(part 1 of 2)
# Autodesk Inventor assembly: Functioning Test Chasis
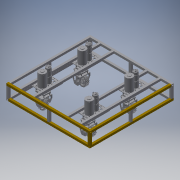
[picture p0: Inventor's stored thumbnail of the model, 180x180]
Saved by Autodesk Inventor 2019 (Build 230136000, 136)
## iProperties
has-driver: True
driver-type: 1
motor-type: 0
driver-port1: 0
driver-port2: -1
driver-isCan: False
driver-lowerLimit: 0.0
driver-upperLimit: 0.0
driver-inputGear: 0.0
driver-outputGear: 0.0
driver-hasBrake: False
has-wheel: True
wheel-type: 3
wheel-isDriveWheel: True
wheel-frictionLevel: 1
has-pneumatic: False
has-elevator: False
num-sensors: 0
has-driver: False
driver-port1: 1
robot-name: Chasis
robot-weight-kg: 222.26052856445312
robot-prefer-metric: False
robot-driveTrainType: 1
Created: 2019-01-14
Part Number: Functioning Test Chasis
Document SubType Name: Assembly
Designer: josh
Author: josh
## Documents named in this file (37)
- D:\Synthesis Robots\Epsilon\Functioning Test Chasis.iam
- D:\Synthesis Robots\Epsilon\Chasis.iam
- D:\Synthesis Robots\Epsilon\functioning swerve drive.iam
- D:\Synthesis Robots\Epsilon\4 in HiGrip Wheel.iam
- D:\Synthesis Robots\Epsilon\FR6ZZ-L Hex Bearing.ipt
- D:\Synthesis Robots\Epsilon\375 Hex Output Shaft Rev 2.ipt
- D:\Synthesis Robots\Epsilon\375 Hex Hub.ipt
- D:\Synthesis Robots\Epsilon\10-24 Hex Washer Rolling x 3-4_93882A213.ipt
- D:\Synthesis Robots\Epsilon\125x443 spacer SPS-0750-0443-0125.ipt
- D:\Synthesis Robots\Epsilon\375 E-klip - Mcm 97431A320_97431A320.ipt
- D:\Synthesis Robots\Epsilon\20t 1-25mod bevel gear.ipt
- D:\Synthesis Robots\Epsilon\40t 1-25mod bevel gear.ipt
- D:\Synthesis Robots\Epsilon\AMS C Housing Rev 2.ipt
- D:\Synthesis Robots\Epsilon\10-32 Nylock Nut 1_90631A411.ipt
- D:\Synthesis Robots\Epsilon\10-32x1250_shcs.ipt
- D:\Synthesis Robots\Epsilon\620x215 alum spacer 83062 K-S.ipt
- D:\Synthesis Robots\Epsilon\Bevel Input Shaft.ipt
- D:\Synthesis Robots\Epsilon\FR8ZZ Bearing_smart.ipt
- D:\Synthesis Robots\Epsilon\FR6ZZ Bearing_smart.ipt
- D:\Synthesis Robots\Epsilon\12T CIM Shaft.ipt
- D:\Synthesis Robots\Epsilon\Gear Plate.ipt
- D:\Synthesis Robots\Epsilon\40T 20dp 375h_Inch - Spur gear 20DP 40T 14.5PA .372FW ---S40N3.0H2.0L0.25N.ipt
- D:\Synthesis Robots\Epsilon\500 Washer am-1001.ipt
- D:\Synthesis Robots\Epsilon\10-32x0625_shcs_HX-SHCS 0.19-32x1.375x1-C.ipt
- D:\Synthesis Robots\Epsilon\1100x215 alum spacer 83062 K-S.ipt
- D:\Synthesis Robots\Epsilon\10-32 Nylock Nut.ipt
- D:\Synthesis Robots\Epsilon\10-32x1750_shcs_HX-SHCS 0.19-32x1.375x1-C.ipt
- D:\Synthesis Robots\Epsilon\Bearing Plate.ipt
- D:\Synthesis Robots\Epsilon\40T Sleeve Gear REV2.ipt
- D:\Synthesis Robots\Epsilon\VEX 217-2736 0500 Collar Clamp.ipt
- D:\Synthesis Robots\Epsilon\CIM Motor SW.ipt
- D:\Synthesis Robots\Epsilon\Motor Mount Plate Rev 2.ipt
- D:\Synthesis Robots\Epsilon\48T 10mm bore gear.ipt
- D:\Synthesis Robots\Epsilon\PG-71.ipt
- D:\Synthesis Robots\Epsilon\SHCS M4x10_91290A187.ipt
- D:\Synthesis Robots\Epsilon\438x406 spacer 13RS100043.ipt
- D:\Synthesis Robots\Epsilon\375 External Self Locking Ring_98430A134.ipt
## Components (274 placed, 36 different names)
1. Chasis:1 [sub-assembly] — Mate:253, Flush:23, Mate:254, Mate:505, Flush:46, Mate:506, Mate:507, Flush:47, Mate:508, Mate:634, Flush:59, Mate:635
2. functioning swerve drive:1 [sub-assembly]
3. FR6ZZ-L Hex Bearing:3
4. FR6ZZ-L Hex Bearing:4
5. 375 Hex Output Shaft Rev 2:2
6. 375 Hex Hub:2
7. 10-24 Hex Washer Rolling x 3-4_93882A213:7
8. 10-24 Hex Washer Rolling x 3-4_93882A213:8
9. 10-24 Hex Washer Rolling x 3-4_93882A213:9
10. 10-24 Hex Washer Rolling x 3-4_93882A213:10
11. 10-24 Hex Washer Rolling x 3-4_93882A213:11
12. 10-24 Hex Washer Rolling x 3-4_93882A213:12
13. 125x443 spacer SPS-0750-0443-0125:2
14. 375 E-klip - Mcm 97431A320_97431A320:2
15. 20t 1-25mod bevel gear:2
16. 40t 1-25mod bevel gear:2
17. AMS C Housing Rev 2:2
18. 10-32 Nylock Nut 1_90631A411:5
19. 10-32 Nylock Nut 1_90631A411:6
20. 10-32 Nylock Nut 1_90631A411:7
21. 10-32 Nylock Nut 1_90631A411:8
22. 10-32x1250_shcs:5
23. 10-32x1250_shcs:6
24. 10-32x1250_shcs:7
25. 10-32x1250_shcs:8
26. 620x215 alum spacer 83062 K-S:5
27. 620x215 alum spacer 83062 K-S:6
28. 620x215 alum spacer 83062 K-S:7
29. 620x215 alum spacer 83062 K-S:8
30. Bevel Input Shaft:2
31. FR8ZZ Bearing_smart:2
32. FR6ZZ Bearing_smart:3
33. 12T CIM Shaft:2
34. Gear Plate:2
35. 40T 20dp 375h_Inch - Spur gear 20DP 40T 14.5PA .372FW ---S40N3.0H2.0L0.25N:2
36. 500 Washer am-1001:3
37. 500 Washer am-1001:4
38. FR6ZZ Bearing_smart:4
39. 10-32x0625_shcs_HX-SHCS 0.19-32x1.375x1-C:7
40. 10-32x0625_shcs_HX-SHCS 0.19-32x1.375x1-C:8
41. 10-32x0625_shcs_HX-SHCS 0.19-32x1.375x1-C:9
42. 10-32x0625_shcs_HX-SHCS 0.19-32x1.375x1-C:10
43. 1100x215 alum spacer 83062 K-S:5
44. 10-32 Nylock Nut:5
45. 10-32x1750_shcs_HX-SHCS 0.19-32x1.375x1-C:5
46. 1100x215 alum spacer 83062 K-S:6
47. 1100x215 alum spacer 83062 K-S:7
48. 1100x215 alum spacer 83062 K-S:8
49. 10-32x1750_shcs_HX-SHCS 0.19-32x1.375x1-C:6
50. 10-32x1750_shcs_HX-SHCS 0.19-32x1.375x1-C:7
51. 10-32x1750_shcs_HX-SHCS 0.19-32x1.375x1-C:8
52. 10-32 Nylock Nut:6
53. 10-32 Nylock Nut:7
54. 10-32 Nylock Nut:8
55. Bearing Plate:2
56. 40T Sleeve Gear REV2:2
57. VEX 217-2736 0500 Collar Clamp:2
58. CIM Motor SW:2
59. Motor Mount Plate Rev 2:2 — Mate:253, Flush:23, Mate:254
60. 48T 10mm bore gear:2
61. 10-32x0625_shcs_HX-SHCS 0.19-32x1.375x1-C:11
62. 10-32x0625_shcs_HX-SHCS 0.19-32x1.375x1-C:12
63. PG-71:2
64. SHCS M4x10_91290A187:5
65. SHCS M4x10_91290A187:6
66. SHCS M4x10_91290A187:7
67. SHCS M4x10_91290A187:8
68. 438x406 spacer 13RS100043:2
69. 375 External Self Locking Ring_98430A134:2
70. 4 in HiGrip Wheel:2 [sub-assembly]
71. FR6ZZ-L Hex Bearing:5
72. FR6ZZ-L Hex Bearing:6
73. 375 Hex Output Shaft Rev 2:3
74. 375 Hex Hub:3
75. 10-24 Hex Washer Rolling x 3-4_93882A213:13
76. 10-24 Hex Washer Rolling x 3-4_93882A213:14
77. 10-24 Hex Washer Rolling x 3-4_93882A213:15
78. 10-24 Hex Washer Rolling x 3-4_93882A213:16
79. 10-24 Hex Washer Rolling x 3-4_93882A213:17
80. 10-24 Hex Washer Rolling x 3-4_93882A213:18
81. 125x443 spacer SPS-0750-0443-0125:3
82. 375 E-klip - Mcm 97431A320_97431A320:3
83. 20t 1-25mod bevel gear:3
84. 40t 1-25mod bevel gear:3
85. AMS C Housing Rev 2:3
86. 10-32 Nylock Nut 1_90631A411:9
87. 10-32 Nylock Nut 1_90631A411:10
88. 10-32 Nylock Nut 1_90631A411:11
89. 10-32 Nylock Nut 1_90631A411:12
90. 10-32x1250_shcs:9
91. 10-32x1250_shcs:10
92. 10-32x1250_shcs:11
93. 10-32x1250_shcs:12
94. 620x215 alum spacer 83062 K-S:9
95. 620x215 alum spacer 83062 K-S:10
96. 620x215 alum spacer 83062 K-S:11
97. 620x215 alum spacer 83062 K-S:12
98. Bevel Input Shaft:3
99. FR8ZZ Bearing_smart:3
100. FR6ZZ Bearing_smart:5
101. 12T CIM Shaft:3
102. Gear Plate:3
103. 40T 20dp 375h_Inch - Spur gear 20DP 40T 14.5PA .372FW ---S40N3.0H2.0L0.25N:3
104. 500 Washer am-1001:5
105. 500 Washer am-1001:6
106. FR6ZZ Bearing_smart:6
107. 10-32x0625_shcs_HX-SHCS 0.19-32x1.375x1-C:13
108. 10-32x0625_shcs_HX-SHCS 0.19-32x1.375x1-C:14
109. 10-32x0625_shcs_HX-SHCS 0.19-32x1.375x1-C:15
110. 10-32x0625_shcs_HX-SHCS 0.19-32x1.375x1-C:16
111. 1100x215 alum spacer 83062 K-S:9
112. 10-32 Nylock Nut:9
113. 10-32x1750_shcs_HX-SHCS 0.19-32x1.375x1-C:9
114. 1100x215 alum spacer 83062 K-S:10
115. 1100x215 alum spacer 83062 K-S:11
116. 1100x215 alum spacer 83062 K-S:12
117. 10-32x1750_shcs_HX-SHCS 0.19-32x1.375x1-C:10
118. 10-32x1750_shcs_HX-SHCS 0.19-32x1.375x1-C:11
119. 10-32x1750_shcs_HX-SHCS 0.19-32x1.375x1-C:12
120. 10-32 Nylock Nut:10
121. 10-32 Nylock Nut:11
122. 10-32 Nylock Nut:12
123. Bearing Plate:3
124. 40T Sleeve Gear REV2:3
125. VEX 217-2736 0500 Collar Clamp:3
126. CIM Motor SW:3
127. Motor Mount Plate Rev 2:3 — Mate:505, Flush:46, Mate:506
128. 48T 10mm bore gear:3
129. 10-32x0625_shcs_HX-SHCS 0.19-32x1.375x1-C:17
130. 10-32x0625_shcs_HX-SHCS 0.19-32x1.375x1-C:18
131. PG-71:3
132. SHCS M4x10_91290A187:9
133. SHCS M4x10_91290A187:10
134. SHCS M4x10_91290A187:11
135. SHCS M4x10_91290A187:12
136. 438x406 spacer 13RS100043:3
137. 375 External Self Locking Ring_98430A134:3
138. 4 in HiGrip Wheel:3 [sub-assembly]
139. FR6ZZ-L Hex Bearing:7
140. FR6ZZ-L Hex Bearing:8
141. 375 Hex Output Shaft Rev 2:4
142. 375 Hex Hub:4
143. 10-24 Hex Washer Rolling x 3-4_93882A213:19
144. 10-24 Hex Washer Rolling x 3-4_93882A213:20
145. 10-24 Hex Washer Rolling x 3-4_93882A213:21
146. 10-24 Hex Washer Rolling x 3-4_93882A213:22
147. 10-24 Hex Washer Rolling x 3-4_93882A213:23
148. 10-24 Hex Washer Rolling x 3-4_93882A213:24
149. 125x443 spacer SPS-0750-0443-0125:4
150. 375 E-klip - Mcm 97431A320_97431A320:4
151. 20t 1-25mod bevel gear:4
152. 40t 1-25mod bevel gear:4
153. AMS C Housing Rev 2:4
154. 10-32 Nylock Nut 1_90631A411:13
155. 10-32 Nylock Nut 1_90631A411:14
156. 10-32 Nylock Nut 1_90631A411:15
157. 10-32 Nylock Nut 1_90631A411:16
158. 10-32x1250_shcs:13
159. 10-32x1250_shcs:14
160. 10-32x1250_shcs:15
161. 10-32x1250_shcs:16
162. 620x215 alum spacer 83062 K-S:13
163. 620x215 alum spacer 83062 K-S:14
164. 620x215 alum spacer 83062 K-S:15
165. 620x215 alum spacer 83062 K-S:16
166. Bevel Input Shaft:4
167. FR8ZZ Bearing_smart:4
168. FR6ZZ Bearing_smart:7
169. 12T CIM Shaft:4
170. Gear Plate:4
171. 40T 20dp 375h_Inch - Spur gear 20DP 40T 14.5PA .372FW ---S40N3.0H2.0L0.25N:4
172. 500 Washer am-1001:7
173. 500 Washer am-1001:8
174. FR6ZZ Bearing_smart:8
175. 10-32x0625_shcs_HX-SHCS 0.19-32x1.375x1-C:19
176. 10-32x0625_shcs_HX-SHCS 0.19-32x1.375x1-C:20
177. 10-32x0625_shcs_HX-SHCS 0.19-32x1.375x1-C:21
178. 10-32x0625_shcs_HX-SHCS 0.19-32x1.375x1-C:22
179. 1100x215 alum spacer 83062 K-S:13
180. 10-32 Nylock Nut:13
181. 10-32x1750_shcs_HX-SHCS 0.19-32x1.375x1-C:13
182. 1100x215 alum spacer 83062 K-S:14
183. 1100x215 alum spacer 83062 K-S:15
184. 1100x215 alum spacer 83062 K-S:16
185. 10-32x1750_shcs_HX-SHCS 0.19-32x1.375x1-C:14
186. 10-32x1750_shcs_HX-SHCS 0.19-32x1.375x1-C:15
187. 10-32x1750_shcs_HX-SHCS 0.19-32x1.375x1-C:16
188. 10-32 Nylock Nut:14
189. 10-32 Nylock Nut:15
190. 10-32 Nylock Nut:16
191. Bearing Plate:4
192. 40T Sleeve Gear REV2:4
193. VEX 217-2736 0500 Collar Clamp:4
194. CIM Motor SW:4
195. Motor Mount Plate Rev 2:4 — Mate:507, Flush:47, Mate:508
196. 48T 10mm bore gear:4
197. 10-32x0625_shcs_HX-SHCS 0.19-32x1.375x1-C:23
198. 10-32x0625_shcs_HX-SHCS 0.19-32x1.375x1-C:24
199. PG-71:4
200. SHCS M4x10_91290A187:13
201. SHCS M4x10_91290A187:14
202. SHCS M4x10_91290A187:15
203. SHCS M4x10_91290A187:16
204. 438x406 spacer 13RS100043:4
205. 375 External Self Locking Ring_98430A134:4
206. 4 in HiGrip Wheel:4 [sub-assembly]
207. FR6ZZ-L Hex Bearing:9
208. FR6ZZ-L Hex Bearing:10
209. 375 Hex Output Shaft Rev 2:5
210. 375 Hex Hub:5
211. 10-24 Hex Washer Rolling x 3-4_93882A213:25
212. 10-24 Hex Washer Rolling x 3-4_93882A213:26
213. 10-24 Hex Washer Rolling x 3-4_93882A213:27
214. 10-24 Hex Washer Rolling x 3-4_93882A213:28
215. 10-24 Hex Washer Rolling x 3-4_93882A213:29
216. 10-24 Hex Washer Rolling x 3-4_93882A213:30
217. 125x443 spacer SPS-0750-0443-0125:5
218. 375 E-klip - Mcm 97431A320_97431A320:5
219. 20t 1-25mod bevel gear:5
220. 40t 1-25mod bevel gear:5
221. AMS C Housing Rev 2:5
222. 10-32 Nylock Nut 1_90631A411:17
223. 10-32 Nylock Nut 1_90631A411:18
224. 10-32 Nylock Nut 1_90631A411:19
225. 10-32 Nylock Nut 1_90631A411:20
226. 10-32x1250_shcs:17
227. 10-32x1250_shcs:18
228. 10-32x1250_shcs:19
229. 10-32x1250_shcs:20
230. 620x215 alum spacer 83062 K-S:17
231. 620x215 alum spacer 83062 K-S:18
232. 620x215 alum spacer 83062 K-S:19
233. 620x215 alum spacer 83062 K-S:20
234. Bevel Input Shaft:5
235. FR8ZZ Bearing_smart:5
236. FR6ZZ Bearing_smart:9
237. 12T CIM Shaft:5
238. Gear Plate:5
239. 40T 20dp 375h_Inch - Spur gear 20DP 40T 14.5PA .372FW ---S40N3.0H2.0L0.25N:5
240. 500 Washer am-1001:9
241. 500 Washer am-1001:10
242. FR6ZZ Bearing_smart:10
243. 10-32x0625_shcs_HX-SHCS 0.19-32x1.375x1-C:25
244. 10-32x0625_shcs_HX-SHCS 0.19-32x1.375x1-C:26
245. 10-32x0625_shcs_HX-SHCS 0.19-32x1.375x1-C:27
246. 10-32x0625_shcs_HX-SHCS 0.19-32x1.375x1-C:28
247. 1100x215 alum spacer 83062 K-S:17
248. 10-32 Nylock Nut:17
249. 10-32x1750_shcs_HX-SHCS 0.19-32x1.375x1-C:17
250. 1100x215 alum spacer 83062 K-S:18
251. 1100x215 alum spacer 83062 K-S:19
252. 1100x215 alum spacer 83062 K-S:20
253. 10-32x1750_shcs_HX-SHCS 0.19-32x1.375x1-C:18
254. 10-32x1750_shcs_HX-SHCS 0.19-32x1.375x1-C:19
255. 10-32x1750_shcs_HX-SHCS 0.19-32x1.375x1-C:20
256. 10-32 Nylock Nut:18
257. 10-32 Nylock Nut:19
258. 10-32 Nylock Nut:20
259. Bearing Plate:5
260. 40T Sleeve Gear REV2:5
261. VEX 217-2736 0500 Collar Clamp:5
262. CIM Motor SW:5
263. Motor Mount Plate Rev 2:5 — Mate:634, Flush:59, Mate:635
264. 48T 10mm bore gear:5
265. 10-32x0625_shcs_HX-SHCS 0.19-32x1.375x1-C:29
266. 10-32x0625_shcs_HX-SHCS 0.19-32x1.375x1-C:30
267. PG-71:5
268. SHCS M4x10_91290A187:17
269. SHCS M4x10_91290A187:18
270. SHCS M4x10_91290A187:19
271. SHCS M4x10_91290A187:20
272. 438x406 spacer 13RS100043:5
273. 375 External Self Locking Ring_98430A134:5
274. 4 in HiGrip Wheel:5 [sub-assembly]
## Relationships (592: Mate 508, Flush 48, RevoluteJoint 28, RelateRotation 8)
- [Mate]: 375 Hex Hub:2 ↔ 10-24 Hex Washer Rolling x 3-4_93882A213:12
- [Mate]: 375 Hex Hub:2 ↔ 10-24 Hex Washer Rolling x 3-4_93882A213:7
- [Mate]: 375 Hex Hub:2 ↔ 10-24 Hex Washer Rolling x 3-4_93882A213:11
- [Mate]: 375 Hex Hub:2 ↔ 10-24 Hex Washer Rolling x 3-4_93882A213:10
- [Mate]: 375 Hex Hub:2 ↔ 10-24 Hex Washer Rolling x 3-4_93882A213:9
- [Mate]: 375 Hex Hub:2 ↔ 10-24 Hex Washer Rolling x 3-4_93882A213:8
- [Mate]: 375 Hex Hub:2 ↔ 10-24 Hex Washer Rolling x 3-4_93882A213:8
- [Mate]: 375 Hex Hub:2 ↔ 10-24 Hex Washer Rolling x 3-4_93882A213:10
- [Mate]: 375 Hex Hub:2 ↔ 10-24 Hex Washer Rolling x 3-4_93882A213:9
- [Mate]: 375 Hex Hub:2 ↔ 10-24 Hex Washer Rolling x 3-4_93882A213:7
- [Mate]: 375 Hex Hub:2 ↔ 10-24 Hex Washer Rolling x 3-4_93882A213:12
- [Mate]: 375 Hex Hub:2 ↔ 10-24 Hex Washer Rolling x 3-4_93882A213:11
- [Mate]: 375 Hex Output Shaft Rev 2:2 ↔ 375 Hex Hub:2
- [Mate]: 375 Hex Output Shaft Rev 2:2 ↔ 375 Hex Hub:2
- [Mate]: FR6ZZ-L Hex Bearing:3 ↔ 375 Hex Output Shaft Rev 2:2
- [Mate]: FR6ZZ-L Hex Bearing:3 ↔ 375 Hex Output Shaft Rev 2:2
- [Mate]: 375 Hex Output Shaft Rev 2:2 ↔ 40t 1-25mod bevel gear:2
- [Mate]: 375 Hex Output Shaft Rev 2:2 ↔ 40t 1-25mod bevel gear:2
- [RevoluteJoint]: FR6ZZ-L Hex Bearing:4 ↔ AMS C Housing Rev 2:2
- [RevoluteJoint]: FR6ZZ-L Hex Bearing:3 ↔ AMS C Housing Rev 2:2
- [Mate]: FR6ZZ-L Hex Bearing:3 ↔ 125x443 spacer SPS-0750-0443-0125:2
- [Mate]: FR6ZZ-L Hex Bearing:3 ↔ 125x443 spacer SPS-0750-0443-0125:2
- [Mate]: 375 Hex Output Shaft Rev 2:2 ↔ 375 E-klip - Mcm 97431A320_97431A320:2
- [Mate]: 375 Hex Output Shaft Rev 2:2 ↔ 375 E-klip - Mcm 97431A320_97431A320:2
- [Mate]: 375 Hex Hub:2 ↔ 125x443 spacer SPS-0750-0443-0125:2
- [Flush]: FR6ZZ-L Hex Bearing:3 ↔ 375 Hex Output Shaft Rev 2:2
- [RevoluteJoint]: 10-32 Nylock Nut 1_90631A411:5 ↔ 10-32x1250_shcs:7
- [RevoluteJoint]: 10-32 Nylock Nut 1_90631A411:6 ↔ 10-32x1250_shcs:8
- [RevoluteJoint]: 10-32 Nylock Nut 1_90631A411:8 ↔ 10-32x1250_shcs:6
- [RevoluteJoint]: 10-32 Nylock Nut 1_90631A411:7 ↔ 10-32x1250_shcs:5
- [Mate]: 10-32x1250_shcs:6 ↔ Gear Plate:2
- [Mate]: 10-32x1250_shcs:6 ↔ 620x215 alum spacer 83062 K-S:6
- [Flush]: 10-32x1250_shcs:6 ↔ Gear Plate:2
- [Mate]: 620x215 alum spacer 83062 K-S:6 ↔ Gear Plate:2
- [Mate]: 10-32x1250_shcs:5 ↔ Gear Plate:2
- [Mate]: 10-32x1250_shcs:5 ↔ 620x215 alum spacer 83062 K-S:5
- [Flush]: 10-32x1250_shcs:5 ↔ Gear Plate:2
- [Mate]: 620x215 alum spacer 83062 K-S:5 ↔ Gear Plate:2
- [Mate]: 10-32x1250_shcs:7 ↔ Gear Plate:2
- [Flush]: 10-32x1250_shcs:7 ↔ Gear Plate:2
- [Mate]: 10-32x1250_shcs:7 ↔ 620x215 alum spacer 83062 K-S:7
- [Mate]: 620x215 alum spacer 83062 K-S:7 ↔ Gear Plate:2
- [Mate]: 10-32x1250_shcs:8 ↔ 620x215 alum spacer 83062 K-S:8
- [Flush]: 10-32x1250_shcs:8 ↔ Gear Plate:2
- [Mate]: 10-32x1250_shcs:8 ↔ Gear Plate:2
- [Mate]: 620x215 alum spacer 83062 K-S:8 ↔ Gear Plate:2
- [Mate]: FR8ZZ Bearing_smart:2 ↔ 12T CIM Shaft:2
- [Mate]: FR8ZZ Bearing_smart:2 ↔ 12T CIM Shaft:2
- [Mate]: 12T CIM Shaft:2 ↔ Gear Plate:2
- [Mate]: Bevel Input Shaft:2 ↔ FR6ZZ Bearing_smart:3
- [Mate]: Bevel Input Shaft:2 ↔ 500 Washer am-1001:3
- [Mate]: Bevel Input Shaft:2 ↔ 40T 20dp 375h_Inch - Spur gear 20DP 40T 14.5PA .372FW ---S40N3.0H2.0L0.25N:2
- [Mate]: Bevel Input Shaft:2 ↔ 40T 20dp 375h_Inch - Spur gear 20DP 40T 14.5PA .372FW ---S40N3.0H2.0L0.25N:2
- [Flush]: Bevel Input Shaft:2 ↔ 40T 20dp 375h_Inch - Spur gear 20DP 40T 14.5PA .372FW ---S40N3.0H2.0L0.25N:2
- [Mate]: Bevel Input Shaft:2 ↔ 500 Washer am-1001:4
- [Mate]: Bevel Input Shaft:2 ↔ FR6ZZ Bearing_smart:4
- [Mate]: 500 Washer am-1001:4 ↔ FR6ZZ Bearing_smart:4
- [Mate]: Bevel Input Shaft:2 ↔ 500 Washer am-1001:4
- [Flush]: Bevel Input Shaft:2 ↔ 500 Washer am-1001:3
- [Mate]: Gear Plate:2 ↔ FR6ZZ Bearing_smart:4
- [Mate]: Gear Plate:2 ↔ FR6ZZ Bearing_smart:4
- [RevoluteJoint]: 20t 1-25mod bevel gear:2 ↔ Bevel Input Shaft:2
- [Mate]: Gear Plate:2 ↔ 10-32x0625_shcs_HX-SHCS 0.19-32x1.375x1-C:9
- [Flush]: Gear Plate:2 ↔ 10-32x0625_shcs_HX-SHCS 0.19-32x1.375x1-C:9
- [Mate]: Gear Plate:2 ↔ 10-32x0625_shcs_HX-SHCS 0.19-32x1.375x1-C:8
- [Flush]: Gear Plate:2 ↔ 10-32x0625_shcs_HX-SHCS 0.19-32x1.375x1-C:8
- [Mate]: Gear Plate:2 ↔ 10-32x0625_shcs_HX-SHCS 0.19-32x1.375x1-C:7
- [Flush]: Gear Plate:2 ↔ 10-32x0625_shcs_HX-SHCS 0.19-32x1.375x1-C:7
- [Mate]: Gear Plate:2 ↔ 10-32x0625_shcs_HX-SHCS 0.19-32x1.375x1-C:10
- [Flush]: Gear Plate:2 ↔ 10-32x0625_shcs_HX-SHCS 0.19-32x1.375x1-C:10
- [Mate]: FR6ZZ Bearing_smart:3 ↔ 500 Washer am-1001:3
- [Mate]: AMS C Housing Rev 2:2 ↔ 10-32x1250_shcs:6
- [Mate]: AMS C Housing Rev 2:2 ↔ 10-32x1250_shcs:5
- [Mate]: AMS C Housing Rev 2:2 ↔ FR6ZZ Bearing_smart:3
- [Mate]: AMS C Housing Rev 2:2 ↔ FR8ZZ Bearing_smart:2
- [Mate]: 10-32x0625_shcs_HX-SHCS 0.19-32x1.375x1-C:9 ↔ 40T Sleeve Gear REV2:2
- [Mate]: 10-32x0625_shcs_HX-SHCS 0.19-32x1.375x1-C:10 ↔ 40T Sleeve Gear REV2:2
- [Mate]: 10-32x0625_shcs_HX-SHCS 0.19-32x1.375x1-C:7 ↔ 40T Sleeve Gear REV2:2
- [Mate]: 10-32x0625_shcs_HX-SHCS 0.19-32x1.375x1-C:8 ↔ 40T Sleeve Gear REV2:2
- [Mate]: 12T CIM Shaft:2 ↔ 40T Sleeve Gear REV2:2
- [Mate]: Gear Plate:2 ↔ 40T Sleeve Gear REV2:2
- [Mate]: 10-32 Nylock Nut:5 ↔ 10-32x1750_shcs_HX-SHCS 0.19-32x1.375x1-C:5
- [Mate]: 10-32x1750_shcs_HX-SHCS 0.19-32x1.375x1-C:8 ↔ 10-32 Nylock Nut:6
- [Mate]: 10-32x1750_shcs_HX-SHCS 0.19-32x1.375x1-C:7 ↔ 10-32 Nylock Nut:8
- [Mate]: 10-32x1750_shcs_HX-SHCS 0.19-32x1.375x1-C:6 ↔ 10-32 Nylock Nut:7
- [Mate]: 1100x215 alum spacer 83062 K-S:7 ↔ 10-32x1750_shcs_HX-SHCS 0.19-32x1.375x1-C:7
- [Mate]: 10-32x1750_shcs_HX-SHCS 0.19-32x1.375x1-C:7 ↔ Bearing Plate:2
- [Mate]: 10-32x1750_shcs_HX-SHCS 0.19-32x1.375x1-C:7 ↔ Bearing Plate:2
- [Mate]: 1100x215 alum spacer 83062 K-S:6 ↔ 10-32x1750_shcs_HX-SHCS 0.19-32x1.375x1-C:8
- [Mate]: 10-32x1750_shcs_HX-SHCS 0.19-32x1.375x1-C:8 ↔ Bearing Plate:2
- [Mate]: 1100x215 alum spacer 83062 K-S:6 ↔ Bearing Plate:2
- [Mate]: 10-32x1750_shcs_HX-SHCS 0.19-32x1.375x1-C:8 ↔ Bearing Plate:2
- [Mate]: 10-32 Nylock Nut:6 ↔ Motor Mount Plate Rev 2:2
- [Mate]: 1100x215 alum spacer 83062 K-S:7 ↔ Bearing Plate:2
- [Mate]: 10-32 Nylock Nut:8 ↔ Motor Mount Plate Rev 2:2
- [Mate]: 10-32x1750_shcs_HX-SHCS 0.19-32x1.375x1-C:5 ↔ Bearing Plate:2
- [Mate]: 10-32 Nylock Nut:5 ↔ 10-32x1750_shcs_HX-SHCS 0.19-32x1.375x1-C:5
- [Mate]: 10-32 Nylock Nut:5 ↔ Motor Mount Plate Rev 2:2
- [Mate]: 10-32x1750_shcs_HX-SHCS 0.19-32x1.375x1-C:5 ↔ Bearing Plate:2
- [Mate]: 1100x215 alum spacer 83062 K-S:5 ↔ 10-32x1750_shcs_HX-SHCS 0.19-32x1.375x1-C:5
- [Mate]: 1100x215 alum spacer 83062 K-S:5 ↔ Bearing Plate:2
- [Mate]: 10-32x1750_shcs_HX-SHCS 0.19-32x1.375x1-C:6 ↔ Bearing Plate:2
- [Mate]: 10-32x1750_shcs_HX-SHCS 0.19-32x1.375x1-C:6 ↔ Bearing Plate:2
- [Mate]: 1100x215 alum spacer 83062 K-S:8 ↔ 10-32x1750_shcs_HX-SHCS 0.19-32x1.375x1-C:6
- [Mate]: 1100x215 alum spacer 83062 K-S:8 ↔ Bearing Plate:2
- [Mate]: 10-32 Nylock Nut:7 ↔ Motor Mount Plate Rev 2:2
- [Mate]: CIM Motor SW:2 ↔ 10-32x0625_shcs_HX-SHCS 0.19-32x1.375x1-C:12
- [Mate]: Motor Mount Plate Rev 2:2 ↔ 10-32x0625_shcs_HX-SHCS 0.19-32x1.375x1-C:12
- [Mate]: Motor Mount Plate Rev 2:2 ↔ 10-32x0625_shcs_HX-SHCS 0.19-32x1.375x1-C:12
- [Mate]: CIM Motor SW:2 ↔ 10-32x0625_shcs_HX-SHCS 0.19-32x1.375x1-C:11
- [Mate]: Motor Mount Plate Rev 2:2 ↔ 10-32x0625_shcs_HX-SHCS 0.19-32x1.375x1-C:11
- [Mate]: Motor Mount Plate Rev 2:2 ↔ 10-32x0625_shcs_HX-SHCS 0.19-32x1.375x1-C:11
- [Mate]: 12T CIM Shaft:2 ↔ CIM Motor SW:2
- [Mate]: VEX 217-2736 0500 Collar Clamp:2 ↔ CIM Motor SW:2
- [Mate]: VEX 217-2736 0500 Collar Clamp:2 ↔ Motor Mount Plate Rev 2:2
- [Mate]: 12T CIM Shaft:2 ↔ CIM Motor SW:2
- [Mate]: CIM Motor SW:2 ↔ Motor Mount Plate Rev 2:2
- [Mate]: PG-71:2 ↔ 375 External Self Locking Ring_98430A134:2
- [Mate]: 48T 10mm bore gear:2 ↔ PG-71:2
- [Mate]: 10-32x1750_shcs_HX-SHCS 0.19-32x1.375x1-C:5 ↔ Motor Mount Plate Rev 2:2
- [Mate]: 10-32x1750_shcs_HX-SHCS 0.19-32x1.375x1-C:8 ↔ Motor Mount Plate Rev 2:2
- [Mate]: 1100x215 alum spacer 83062 K-S:5 ↔ Motor Mount Plate Rev 2:2
- [Mate]: PG-71:2 ↔ 438x406 spacer 13RS100043:2
- [Mate]: Motor Mount Plate Rev 2:2 ↔ 438x406 spacer 13RS100043:2
- [Mate]: Motor Mount Plate Rev 2:2 ↔ SHCS M4x10_91290A187:6
- [Mate]: Motor Mount Plate Rev 2:2 ↔ SHCS M4x10_91290A187:5
- [Mate]: Motor Mount Plate Rev 2:2 ↔ SHCS M4x10_91290A187:8
- [Mate]: Motor Mount Plate Rev 2:2 ↔ SHCS M4x10_91290A187:7
- [Mate]: Motor Mount Plate Rev 2:2 ↔ SHCS M4x10_91290A187:5
- [Mate]: Motor Mount Plate Rev 2:2 ↔ SHCS M4x10_91290A187:6
- [Mate]: Motor Mount Plate Rev 2:2 ↔ SHCS M4x10_91290A187:8
- [Mate]: Motor Mount Plate Rev 2:2 ↔ SHCS M4x10_91290A187:7
- [Mate]: PG-71:2 ↔ 438x406 spacer 13RS100043:2
- [Mate]: Motor Mount Plate Rev 2:2 ↔ PG-71:2
- [Mate]: 48T 10mm bore gear:2 ↔ 438x406 spacer 13RS100043:2
- [Mate]: PG-71:2 ↔ 375 External Self Locking Ring_98430A134:2
- [RelateRotation] (1 ul): 20t 1-25mod bevel gear:2 ↔ 40t 1-25mod bevel gear:2
- [Mate]: 20t 1-25mod bevel gear:2 ↔ Bevel Input Shaft:2
- [RelateRotation] (1 ul): 40T Sleeve Gear REV2:2 ↔ 48T 10mm bore gear:2
- [Mate]: 48T 10mm bore gear:2 ↔ PG-71:2
- [Mate]: 10-24 Hex Washer Rolling x 3-4_93882A213:12 ↔ 4 in HiGrip Wheel:2
- [Mate]: 10-24 Hex Washer Rolling x 3-4_93882A213:11 ↔ 4 in HiGrip Wheel:2
- [Mate]: 10-24 Hex Washer Rolling x 3-4_93882A213:10 ↔ 4 in HiGrip Wheel:2
- [Mate]: 375 Hex Hub:2 ↔ 4 in HiGrip Wheel:2
- [Mate]: 40t 1-25mod bevel gear:2 ↔ 4 in HiGrip Wheel:2
- Mate:253: Chasis:1 ↔ Motor Mount Plate Rev 2:2
- Flush:23: Chasis:1 ↔ Motor Mount Plate Rev 2:2
- Mate:254 (95.25 mm): Chasis:1 ↔ Motor Mount Plate Rev 2:2
- [Mate]: 375 Hex Hub:3 ↔ 10-24 Hex Washer Rolling x 3-4_93882A213:18
- [Mate]: 375 Hex Hub:3 ↔ 10-24 Hex Washer Rolling x 3-4_93882A213:13
- [Mate]: 375 Hex Hub:3 ↔ 10-24 Hex Washer Rolling x 3-4_93882A213:17
- [Mate]: 375 Hex Hub:3 ↔ 10-24 Hex Washer Rolling x 3-4_93882A213:16
- [Mate]: 375 Hex Hub:3 ↔ 10-24 Hex Washer Rolling x 3-4_93882A213:15
- [Mate]: 375 Hex Hub:3 ↔ 10-24 Hex Washer Rolling x 3-4_93882A213:14
- [Mate]: 375 Hex Hub:3 ↔ 10-24 Hex Washer Rolling x 3-4_93882A213:14
- [Mate]: 375 Hex Hub:3 ↔ 10-24 Hex Washer Rolling x 3-4_93882A213:16
- [Mate]: 375 Hex Hub:3 ↔ 10-24 Hex Washer Rolling x 3-4_93882A213:15
- [Mate]: 375 Hex Hub:3 ↔ 10-24 Hex Washer Rolling x 3-4_93882A213:13
- [Mate]: 375 Hex Hub:3 ↔ 10-24 Hex Washer Rolling x 3-4_93882A213:18
- [Mate]: 375 Hex Hub:3 ↔ 10-24 Hex Washer Rolling x 3-4_93882A213:17
- [Mate]: 375 Hex Output Shaft Rev 2:3 ↔ 375 Hex Hub:3
- [Mate]: 375 Hex Output Shaft Rev 2:3 ↔ 375 Hex Hub:3
- [Mate]: FR6ZZ-L Hex Bearing:5 ↔ 375 Hex Output Shaft Rev 2:3
- [Mate]: FR6ZZ-L Hex Bearing:5 ↔ 375 Hex Output Shaft Rev 2:3
- [Mate]: 375 Hex Output Shaft Rev 2:3 ↔ 40t 1-25mod bevel gear:3
- [Mate]: 375 Hex Output Shaft Rev 2:3 ↔ 40t 1-25mod bevel gear:3
- [RevoluteJoint]: FR6ZZ-L Hex Bearing:6 ↔ AMS C Housing Rev 2:3
- [RevoluteJoint]: FR6ZZ-L Hex Bearing:5 ↔ AMS C Housing Rev 2:3
- [Mate]: FR6ZZ-L Hex Bearing:5 ↔ 125x443 spacer SPS-0750-0443-0125:3
- [Mate]: FR6ZZ-L Hex Bearing:5 ↔ 125x443 spacer SPS-0750-0443-0125:3
- [Mate]: 375 Hex Output Shaft Rev 2:3 ↔ 375 E-klip - Mcm 97431A320_97431A320:3
- [Mate]: 375 Hex Output Shaft Rev 2:3 ↔ 375 E-klip - Mcm 97431A320_97431A320:3
- [Mate]: 375 Hex Hub:3 ↔ 125x443 spacer SPS-0750-0443-0125:3
- [Flush]: FR6ZZ-L Hex Bearing:5 ↔ 375 Hex Output Shaft Rev 2:3
- [RevoluteJoint]: 10-32 Nylock Nut 1_90631A411:9 ↔ 10-32x1250_shcs:11
- [RevoluteJoint]: 10-32 Nylock Nut 1_90631A411:10 ↔ 10-32x1250_shcs:12
- [RevoluteJoint]: 10-32 Nylock Nut 1_90631A411:12 ↔ 10-32x1250_shcs:10
- [RevoluteJoint]: 10-32 Nylock Nut 1_90631A411:11 ↔ 10-32x1250_shcs:9
- [Mate]: 10-32x1250_shcs:10 ↔ Gear Plate:3
- [Mate]: 10-32x1250_shcs:10 ↔ 620x215 alum spacer 83062 K-S:10
- [Flush]: 10-32x1250_shcs:10 ↔ Gear Plate:3
- [Mate]: 620x215 alum spacer 83062 K-S:10 ↔ Gear Plate:3
- [Mate]: 10-32x1250_shcs:9 ↔ Gear Plate:3
- [Mate]: 10-32x1250_shcs:9 ↔ 620x215 alum spacer 83062 K-S:9
- [Flush]: 10-32x1250_shcs:9 ↔ Gear Plate:3
- [Mate]: 620x215 alum spacer 83062 K-S:9 ↔ Gear Plate:3
- [Mate]: 10-32x1250_shcs:11 ↔ Gear Plate:3
- [Flush]: 10-32x1250_shcs:11 ↔ Gear Plate:3
- [Mate]: 10-32x1250_shcs:11 ↔ 620x215 alum spacer 83062 K-S:11
- [Mate]: 620x215 alum spacer 83062 K-S:11 ↔ Gear Plate:3
- [Mate]: 10-32x1250_shcs:12 ↔ 620x215 alum spacer 83062 K-S:12
- [Flush]: 10-32x1250_shcs:12 ↔ Gear Plate:3
- [Mate]: 10-32x1250_shcs:12 ↔ Gear Plate:3
- [Mate]: 620x215 alum spacer 83062 K-S:12 ↔ Gear Plate:3
- [Mate]: FR8ZZ Bearing_smart:3 ↔ 12T CIM Shaft:3
- [Mate]: FR8ZZ Bearing_smart:3 ↔ 12T CIM Shaft:3
- [Mate]: 12T CIM Shaft:3 ↔ Gear Plate:3
- [Mate]: Bevel Input Shaft:3 ↔ FR6ZZ Bearing_smart:5
- [Mate]: Bevel Input Shaft:3 ↔ 500 Washer am-1001:5
- [Mate]: Bevel Input Shaft:3 ↔ 40T 20dp 375h_Inch - Spur gear 20DP 40T 14.5PA .372FW ---S40N3.0H2.0L0.25N:3
- [Mate]: Bevel Input Shaft:3 ↔ 40T 20dp 375h_Inch - Spur gear 20DP 40T 14.5PA .372FW ---S40N3.0H2.0L0.25N:3
- [Flush]: Bevel Input Shaft:3 ↔ 40T 20dp 375h_Inch - Spur gear 20DP 40T 14.5PA .372FW ---S40N3.0H2.0L0.25N:3
- [Mate]: Bevel Input Shaft:3 ↔ 500 Washer am-1001:6
- [Mate]: Bevel Input Shaft:3 ↔ FR6ZZ Bearing_smart:6
- [Mate]: 500 Washer am-1001:6 ↔ FR6ZZ Bearing_smart:6
- [Mate]: Bevel Input Shaft:3 ↔ 500 Washer am-1001:6
- [Flush]: Bevel Input Shaft:3 ↔ 500 Washer am-1001:5
- [Mate]: Gear Plate:3 ↔ FR6ZZ Bearing_smart:6
- [Mate]: Gear Plate:3 ↔ FR6ZZ Bearing_smart:6
- [RevoluteJoint]: 20t 1-25mod bevel gear:3 ↔ Bevel Input Shaft:3
- [Mate]: Gear Plate:3 ↔ 10-32x0625_shcs_HX-SHCS 0.19-32x1.375x1-C:15
- [Flush]: Gear Plate:3 ↔ 10-32x0625_shcs_HX-SHCS 0.19-32x1.375x1-C:15
- [Mate]: Gear Plate:3 ↔ 10-32x0625_shcs_HX-SHCS 0.19-32x1.375x1-C:14
- [Flush]: Gear Plate:3 ↔ 10-32x0625_shcs_HX-SHCS 0.19-32x1.375x1-C:14
- [Mate]: Gear Plate:3 ↔ 10-32x0625_shcs_HX-SHCS 0.19-32x1.375x1-C:13
- [Flush]: Gear Plate:3 ↔ 10-32x0625_shcs_HX-SHCS 0.19-32x1.375x1-C:13
- [Mate]: Gear Plate:3 ↔ 10-32x0625_shcs_HX-SHCS 0.19-32x1.375x1-C:16
- [Flush]: Gear Plate:3 ↔ 10-32x0625_shcs_HX-SHCS 0.19-32x1.375x1-C:16
- [Mate]: FR6ZZ Bearing_smart:5 ↔ 500 Washer am-1001:5
- [Mate]: AMS C Housing Rev 2:3 ↔ 10-32x1250_shcs:10
- [Mate]: AMS C Housing Rev 2:3 ↔ 10-32x1250_shcs:9
- [Mate]: AMS C Housing Rev 2:3 ↔ FR6ZZ Bearing_smart:5
- [Mate]: AMS C Housing Rev 2:3 ↔ FR8ZZ Bearing_smart:3
- [Mate]: 10-32x0625_shcs_HX-SHCS 0.19-32x1.375x1-C:15 ↔ 40T Sleeve Gear REV2:3
- [Mate]: 10-32x0625_shcs_HX-SHCS 0.19-32x1.375x1-C:16 ↔ 40T Sleeve Gear REV2:3
- [Mate]: 10-32x0625_shcs_HX-SHCS 0.19-32x1.375x1-C:13 ↔ 40T Sleeve Gear REV2:3
- [Mate]: 10-32x0625_shcs_HX-SHCS 0.19-32x1.375x1-C:14 ↔ 40T Sleeve Gear REV2:3
- [Mate]: 12T CIM Shaft:3 ↔ 40T Sleeve Gear REV2:3
- [Mate]: Gear Plate:3 ↔ 40T Sleeve Gear REV2:3
- [Mate]: 10-32 Nylock Nut:9 ↔ 10-32x1750_shcs_HX-SHCS 0.19-32x1.375x1-C:9
- [Mate]: 10-32x1750_shcs_HX-SHCS 0.19-32x1.375x1-C:12 ↔ 10-32 Nylock Nut:10
- [Mate]: 10-32x1750_shcs_HX-SHCS 0.19-32x1.375x1-C:11 ↔ 10-32 Nylock Nut:12
- [Mate]: 10-32x1750_shcs_HX-SHCS 0.19-32x1.375x1-C:10 ↔ 10-32 Nylock Nut:11
- [Mate]: 1100x215 alum spacer 83062 K-S:11 ↔ 10-32x1750_shcs_HX-SHCS 0.19-32x1.375x1-C:11
- [Mate]: 10-32x1750_shcs_HX-SHCS 0.19-32x1.375x1-C:11 ↔ Bearing Plate:3
- [Mate]: 10-32x1750_shcs_HX-SHCS 0.19-32x1.375x1-C:11 ↔ Bearing Plate:3
- [Mate]: 1100x215 alum spacer 83062 K-S:10 ↔ 10-32x1750_shcs_HX-SHCS 0.19-32x1.375x1-C:12
- [Mate]: 10-32x1750_shcs_HX-SHCS 0.19-32x1.375x1-C:12 ↔ Bearing Plate:3
- [Mate]: 1100x215 alum spacer 83062 K-S:10 ↔ Bearing Plate:3
- [Mate]: 10-32x1750_shcs_HX-SHCS 0.19-32x1.375x1-C:12 ↔ Bearing Plate:3
- [Mate]: 10-32 Nylock Nut:10 ↔ Motor Mount Plate Rev 2:3
- [Mate]: 1100x215 alum spacer 83062 K-S:11 ↔ Bearing Plate:3
- [Mate]: 10-32 Nylock Nut:12 ↔ Motor Mount Plate Rev 2:3
- [Mate]: 10-32x1750_shcs_HX-SHCS 0.19-32x1.375x1-C:9 ↔ Bearing Plate:3
- [Mate]: 10-32 Nylock Nut:9 ↔ 10-32x1750_shcs_HX-SHCS 0.19-32x1.375x1-C:9
- [Mate]: 10-32 Nylock Nut:9 ↔ Motor Mount Plate Rev 2:3
- [Mate]: 10-32x1750_shcs_HX-SHCS 0.19-32x1.375x1-C:9 ↔ Bearing Plate:3
- [Mate]: 1100x215 alum spacer 83062 K-S:9 ↔ 10-32x1750_shcs_HX-SHCS 0.19-32x1.375x1-C:9
- [Mate]: 1100x215 alum spacer 83062 K-S:9 ↔ Bearing Plate:3
- [Mate]: 10-32x1750_shcs_HX-SHCS 0.19-32x1.375x1-C:10 ↔ Bearing Plate:3
- [Mate]: 10-32x1750_shcs_HX-SHCS 0.19-32x1.375x1-C:10 ↔ Bearing Plate:3
- [Mate]: 1100x215 alum spacer 83062 K-S:12 ↔ 10-32x1750_shcs_HX-SHCS 0.19-32x1.375x1-C:10
- [Mate]: 1100x215 alum spacer 83062 K-S:12 ↔ Bearing Plate:3
- [Mate]: 10-32 Nylock Nut:11 ↔ Motor Mount Plate Rev 2:3
- [Mate]: CIM Motor SW:3 ↔ 10-32x0625_shcs_HX-SHCS 0.19-32x1.375x1-C:18
- [Mate]: Motor Mount Plate Rev 2:3 ↔ 10-32x0625_shcs_HX-SHCS 0.19-32x1.375x1-C:18
- [Mate]: Motor Mount Plate Rev 2:3 ↔ 10-32x0625_shcs_HX-SHCS 0.19-32x1.375x1-C:18
- [Mate]: CIM Motor SW:3 ↔ 10-32x0625_shcs_HX-SHCS 0.19-32x1.375x1-C:17
- [Mate]: Motor Mount Plate Rev 2:3 ↔ 10-32x0625_shcs_HX-SHCS 0.19-32x1.375x1-C:17
- [Mate]: Motor Mount Plate Rev 2:3 ↔ 10-32x0625_shcs_HX-SHCS 0.19-32x1.375x1-C:17
- [Mate]: 12T CIM Shaft:3 ↔ CIM Motor SW:3
- [Mate]: VEX 217-2736 0500 Collar Clamp:3 ↔ CIM Motor SW:3
- [Mate]: VEX 217-2736 0500 Collar Clamp:3 ↔ Motor Mount Plate Rev 2:3
- [Mate]: 12T CIM Shaft:3 ↔ CIM Motor SW:3
- [Mate]: CIM Motor SW:3 ↔ Motor Mount Plate Rev 2:3
- [Mate]: PG-71:3 ↔ 375 External Self Locking Ring_98430A134:3
- [Mate]: 48T 10mm bore gear:3 ↔ PG-71:3
- [Mate]: 10-32x1750_shcs_HX-SHCS 0.19-32x1.375x1-C:9 ↔ Motor Mount Plate Rev 2:3
- [Mate]: 10-32x1750_shcs_HX-SHCS 0.19-32x1.375x1-C:12 ↔ Motor Mount Plate Rev 2:3
- [Mate]: 1100x215 alum spacer 83062 K-S:9 ↔ Motor Mount Plate Rev 2:3
- [Mate]: PG-71:3 ↔ 438x406 spacer 13RS100043:3
- [Mate]: Motor Mount Plate Rev 2:3 ↔ 438x406 spacer 13RS100043:3
- [Mate]: Motor Mount Plate Rev 2:3 ↔ SHCS M4x10_91290A187:10
- [Mate]: Motor Mount Plate Rev 2:3 ↔ SHCS M4x10_91290A187:9
- [Mate]: Motor Mount Plate Rev 2:3 ↔ SHCS M4x10_91290A187:12
- [Mate]: Motor Mount Plate Rev 2:3 ↔ SHCS M4x10_91290A187:11
- [Mate]: Motor Mount Plate Rev 2:3 ↔ SHCS M4x10_91290A187:9
- [Mate]: Motor Mount Plate Rev 2:3 ↔ SHCS M4x10_91290A187:10
- [Mate]: Motor Mount Plate Rev 2:3 ↔ SHCS M4x10_91290A187:12
- [Mate]: Motor Mount Plate Rev 2:3 ↔ SHCS M4x10_91290A187:11
- [Mate]: PG-71:3 ↔ 438x406 spacer 13RS100043:3
- [Mate]: Motor Mount Plate Rev 2:3 ↔ PG-71:3
- [Mate]: 48T 10mm bore gear:3 ↔ 438x406 spacer 13RS100043:3
- [Mate]: PG-71:3 ↔ 375 External Self Locking Ring_98430A134:3
- [RelateRotation] (1 ul): 20t 1-25mod bevel gear:3 ↔ 40t 1-25mod bevel gear:3
- [Mate]: 20t 1-25mod bevel gear:3 ↔ Bevel Input Shaft:3
- [RelateRotation] (1 ul): 40T Sleeve Gear REV2:3 ↔ 48T 10mm bore gear:3
- [Mate]: 48T 10mm bore gear:3 ↔ PG-71:3
- [Mate]: 10-24 Hex Washer Rolling x 3-4_93882A213:18 ↔ 4 in HiGrip Wheel:3
- [Mate]: 10-24 Hex Washer Rolling x 3-4_93882A213:17 ↔ 4 in HiGrip Wheel:3
- [Mate]: 10-24 Hex Washer Rolling x 3-4_93882A213:16 ↔ 4 in HiGrip Wheel:3
- [Mate]: 375 Hex Hub:3 ↔ 4 in HiGrip Wheel:3
- [Mate]: 40t 1-25mod bevel gear:3 ↔ 4 in HiGrip Wheel:3
- [Mate]: 375 Hex Hub:4 ↔ 10-24 Hex Washer Rolling x 3-4_93882A213:24
- [Mate]: 375 Hex Hub:4 ↔ 10-24 Hex Washer Rolling x 3-4_93882A213:19
- [Mate]: 375 Hex Hub:4 ↔ 10-24 Hex Washer Rolling x 3-4_93882A213:23
- [Mate]: 375 Hex Hub:4 ↔ 10-24 Hex Washer Rolling x 3-4_93882A213:22
- [Mate]: 375 Hex Hub:4 ↔ 10-24 Hex Washer Rolling x 3-4_93882A213:21
- [Mate]: 375 Hex Hub:4 ↔ 10-24 Hex Washer Rolling x 3-4_93882A213:20
- [Mate]: 375 Hex Hub:4 ↔ 10-24 Hex Washer Rolling x 3-4_93882A213:20
- [Mate]: 375 Hex Hub:4 ↔ 10-24 Hex Washer Rolling x 3-4_93882A213:22
- [Mate]: 375 Hex Hub:4 ↔ 10-24 Hex Washer Rolling x 3-4_93882A213:21
- [Mate]: 375 Hex Hub:4 ↔ 10-24 Hex Washer Rolling x 3-4_93882A213:19
- [Mate]: 375 Hex Hub:4 ↔ 10-24 Hex Washer Rolling x 3-4_93882A213:24
- [Mate]: 375 Hex Hub:4 ↔ 10-24 Hex Washer Rolling x 3-4_93882A213:23
- [Mate]: 375 Hex Output Shaft Rev 2:4 ↔ 375 Hex Hub:4
- [Mate]: 375 Hex Output Shaft Rev 2:4 ↔ 375 Hex Hub:4
- [Mate]: FR6ZZ-L Hex Bearing:7 ↔ 375 Hex Output Shaft Rev 2:4
- [Mate]: FR6ZZ-L Hex Bearing:7 ↔ 375 Hex Output Shaft Rev 2:4
- [Mate]: 375 Hex Output Shaft Rev 2:4 ↔ 40t 1-25mod bevel gear:4
- [Mate]: 375 Hex Output Shaft Rev 2:4 ↔ 40t 1-25mod bevel gear:4
- [RevoluteJoint]: FR6ZZ-L Hex Bearing:8 ↔ AMS C Housing Rev 2:4
- [RevoluteJoint]: FR6ZZ-L Hex Bearing:7 ↔ AMS C Housing Rev 2:4
- [Mate]: FR6ZZ-L Hex Bearing:7 ↔ 125x443 spacer SPS-0750-0443-0125:4
- [Mate]: FR6ZZ-L Hex Bearing:7 ↔ 125x443 spacer SPS-0750-0443-0125:4
- [Mate]: 375 Hex Output Shaft Rev 2:4 ↔ 375 E-klip - Mcm 97431A320_97431A320:4
- [Mate]: 375 Hex Output Shaft Rev 2:4 ↔ 375 E-klip - Mcm 97431A320_97431A320:4
- [Mate]: 375 Hex Hub:4 ↔ 125x443 spacer SPS-0750-0443-0125:4
- [Flush]: FR6ZZ-L Hex Bearing:7 ↔ 375 Hex Output Shaft Rev 2:4
- [RevoluteJoint]: 10-32 Nylock Nut 1_90631A411:13 ↔ 10-32x1250_shcs:15
- [RevoluteJoint]: 10-32 Nylock Nut 1_90631A411:14 ↔ 10-32x1250_shcs:16
- [RevoluteJoint]: 10-32 Nylock Nut 1_90631A411:16 ↔ 10-32x1250_shcs:14
- [RevoluteJoint]: 10-32 Nylock Nut 1_90631A411:15 ↔ 10-32x1250_shcs:13
- [Mate]: 10-32x1250_shcs:14 ↔ Gear Plate:4
- [Mate]: 10-32x1250_shcs:14 ↔ 620x215 alum spacer 83062 K-S:14
- [Flush]: 10-32x1250_shcs:14 ↔ Gear Plate:4
- [Mate]: 620x215 alum spacer 83062 K-S:14 ↔ Gear Plate:4
- [Mate]: 10-32x1250_shcs:13 ↔ Gear Plate:4
- [Mate]: 10-32x1250_shcs:13 ↔ 620x215 alum spacer 83062 K-S:13
- [Flush]: 10-32x1250_shcs:13 ↔ Gear Plate:4
- [Mate]: 620x215 alum spacer 83062 K-S:13 ↔ Gear Plate:4
- [Mate]: 10-32x1250_shcs:15 ↔ Gear Plate:4
- [Flush]: 10-32x1250_shcs:15 ↔ Gear Plate:4
- [Mate]: 10-32x1250_shcs:15 ↔ 620x215 alum spacer 83062 K-S:15
- [Mate]: 620x215 alum spacer 83062 K-S:15 ↔ Gear Plate:4
- [Mate]: 10-32x1250_shcs:16 ↔ 620x215 alum spacer 83062 K-S:16
- [Flush]: 10-32x1250_shcs:16 ↔ Gear Plate:4
- [Mate]: 10-32x1250_shcs:16 ↔ Gear Plate:4
- [Mate]: 620x215 alum spacer 83062 K-S:16 ↔ Gear Plate:4
- [Mate]: FR8ZZ Bearing_smart:4 ↔ 12T CIM Shaft:4
- [Mate]: FR8ZZ Bearing_smart:4 ↔ 12T CIM Shaft:4
- [Mate]: 12T CIM Shaft:4 ↔ Gear Plate:4
- [Mate]: Bevel Input Shaft:4 ↔ FR6ZZ Bearing_smart:7
- [Mate]: Bevel Input Shaft:4 ↔ 500 Washer am-1001:7
- [Mate]: Bevel Input Shaft:4 ↔ 40T 20dp 375h_Inch - Spur gear 20DP 40T 14.5PA .372FW ---S40N3.0H2.0L0.25N:4
- [Mate]: Bevel Input Shaft:4 ↔ 40T 20dp 375h_Inch - Spur gear 20DP 40T 14.5PA .372FW ---S40N3.0H2.0L0.25N:4
- [Flush]: Bevel Input Shaft:4 ↔ 40T 20dp 375h_Inch - Spur gear 20DP 40T 14.5PA .372FW ---S40N3.0H2.0L0.25N:4
- [Mate]: Bevel Input Shaft:4 ↔ 500 Washer am-1001:8
- [Mate]: Bevel Input Shaft:4 ↔ FR6ZZ Bearing_smart:8
- [Mate]: 500 Washer am-1001:8 ↔ FR6ZZ Bearing_smart:8
- [Mate]: Bevel Input Shaft:4 ↔ 500 Washer am-1001:8
- [Flush]: Bevel Input Shaft:4 ↔ 500 Washer am-1001:7
- [Mate]: Gear Plate:4 ↔ FR6ZZ Bearing_smart:8
- [Mate]: Gear Plate:4 ↔ FR6ZZ Bearing_smart:8
- [RevoluteJoint]: 20t 1-25mod bevel gear:4 ↔ Bevel Input Shaft:4
- [Mate]: Gear Plate:4 ↔ 10-32x0625_shcs_HX-SHCS 0.19-32x1.375x1-C:21
- [Flush]: Gear Plate:4 ↔ 10-32x0625_shcs_HX-SHCS 0.19-32x1.375x1-C:21
- [Mate]: Gear Plate:4 ↔ 10-32x0625_shcs_HX-SHCS 0.19-32x1.375x1-C:20
- [Flush]: Gear Plate:4 ↔ 10-32x0625_shcs_HX-SHCS 0.19-32x1.375x1-C:20
- [Mate]: Gear Plate:4 ↔ 10-32x0625_shcs_HX-SHCS 0.19-32x1.375x1-C:19
- [Flush]: Gear Plate:4 ↔ 10-32x0625_shcs_HX-SHCS 0.19-32x1.375x1-C:19
- [Mate]: Gear Plate:4 ↔ 10-32x0625_shcs_HX-SHCS 0.19-32x1.375x1-C:22
- [Flush]: Gear Plate:4 ↔ 10-32x0625_shcs_HX-SHCS 0.19-32x1.375x1-C:22
- [Mate]: FR6ZZ Bearing_smart:7 ↔ 500 Washer am-1001:7
- [Mate]: AMS C Housing Rev 2:4 ↔ 10-32x1250_shcs:14
- [Mate]: AMS C Housing Rev 2:4 ↔ 10-32x1250_shcs:13
- [Mate]: AMS C Housing Rev 2:4 ↔ FR6ZZ Bearing_smart:7
- [Mate]: AMS C Housing Rev 2:4 ↔ FR8ZZ Bearing_smart:4
- [Mate]: 10-32x0625_shcs_HX-SHCS 0.19-32x1.375x1-C:21 ↔ 40T Sleeve Gear REV2:4
- [Mate]: 10-32x0625_shcs_HX-SHCS 0.19-32x1.375x1-C:22 ↔ 40T Sleeve Gear REV2:4
- [Mate]: 10-32x0625_shcs_HX-SHCS 0.19-32x1.375x1-C:19 ↔ 40T Sleeve Gear REV2:4
- [Mate]: 10-32x0625_shcs_HX-SHCS 0.19-32x1.375x1-C:20 ↔ 40T Sleeve Gear REV2:4
- [Mate]: 12T CIM Shaft:4 ↔ 40T Sleeve Gear REV2:4
- [Mate]: Gear Plate:4 ↔ 40T Sleeve Gear REV2:4
- [Mate]: 10-32 Nylock Nut:13 ↔ 10-32x1750_shcs_HX-SHCS 0.19-32x1.375x1-C:13
- [Mate]: 10-32x1750_shcs_HX-SHCS 0.19-32x1.375x1-C:16 ↔ 10-32 Nylock Nut:14
- [Mate]: 10-32x1750_shcs_HX-SHCS 0.19-32x1.375x1-C:15 ↔ 10-32 Nylock Nut:16
- [Mate]: 10-32x1750_shcs_HX-SHCS 0.19-32x1.375x1-C:14 ↔ 10-32 Nylock Nut:15
- [Mate]: 1100x215 alum spacer 83062 K-S:15 ↔ 10-32x1750_shcs_HX-SHCS 0.19-32x1.375x1-C:15
- [Mate]: 10-32x1750_shcs_HX-SHCS 0.19-32x1.375x1-C:15 ↔ Bearing Plate:4
- [Mate]: 10-32x1750_shcs_HX-SHCS 0.19-32x1.375x1-C:15 ↔ Bearing Plate:4
- [Mate]: 1100x215 alum spacer 83062 K-S:14 ↔ 10-32x1750_shcs_HX-SHCS 0.19-32x1.375x1-C:16
- [Mate]: 10-32x1750_shcs_HX-SHCS 0.19-32x1.375x1-C:16 ↔ Bearing Plate:4